# Autodesk Inventor assembly: Mitutoyo-ManualTurret-4pos-approx
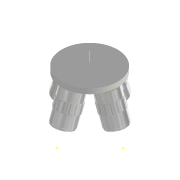
[picture p0: Inventor's stored thumbnail of the model, 180x180]
Saved by Autodesk Inventor 2021 (Build 250183000, 183)
## iProperties
Created: 2022-11-10
Part Number: Mitutoyo-ManualTurret-4pos-approx
Document SubType Name: Assembly
Designer: nvladi
Author: nvladi
## Documents named in this file (3)
- C:\Users\Public\GitHub-public\benchtop-hardware\Benchtop\custom-parts\detection-turret\Mitutoyo-ManualTurret-4pos-approx.iam
- C:\Users\Public\GitHub-public\benchtop-hardware\Benchtop\CAD-model-Inventor2021\library\Mitutoyo\BD-Plan-Apo-approx.ipt
- C:\Users\Public\GitHub-public\benchtop-hardware\Benchtop\custom-parts\detection-turret\TurretMock-4pos.ipt
## Components (5 placed, 2 different names)
1. TurretMock-4pos:1 — Flush:1
2. BD-Plan-Apo-approx:1 — Angle:1
3. BD-Plan-Apo-approx:2
4. BD-Plan-Apo-approx:3
5. BD-Plan-Apo-approx:4
## Component patterns: (4 elements, first: BD-Plan-Apo-approx:1)
## Relationships (2: Angle 1, Flush 1)
- Angle:1 (20 deg): BD-Plan-Apo-approx:1
- Flush:1 (-25 mm): TurretMock-4pos:1
